# Autodesk Inventor assembly: BaffleAssembly2
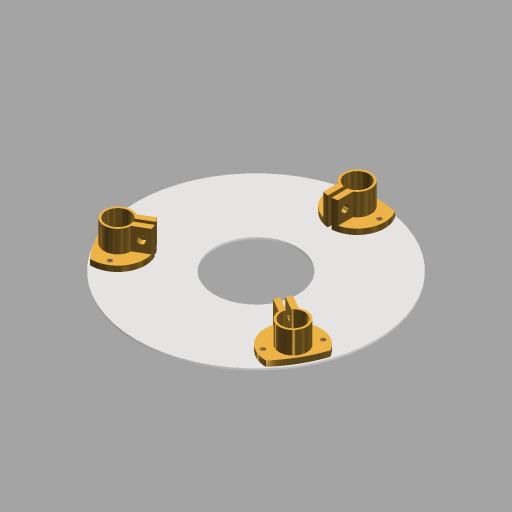
[picture p0: Inventor's stored thumbnail of the model, 512x512]
Saved by Autodesk Inventor 2024 (Build 280153020, 153B)
## iProperties
Created: 2023-10-26
Part Number: BaffleAssembly2
Document SubType Name: Assembly
Designer: schanen
Mass: 44.3536 g
Surface Area: 289.72 cm^2
Volume: 15.1113 cm^3
Density: 2.93513 g/cm^3
Author: schanen
## Documents named in this file (3)
- C:\Users\schanen\Documents\Inventor\LargeTransportDewarInsert2023\BaffleAssembly2.iam
- C:\Users\schanen\Documents\Inventor\LargeTransportDewarInsert2023\Baffle.ipt
- C:\Users\schanen\Documents\Inventor\LargeTransportDewarInsert2023\BaffleClampWithScrew.ipt
## Components (4 placed, 2 different names)
1. Baffle:1 — Mate:1, Mate:2, Mate:3
2. BaffleClampWithScrew:1 [sub-assembly] — Mate:1, Mate:2, Mate:3
3. BaffleClampWithScrew:2 [sub-assembly]
4. BaffleClampWithScrew:3 [sub-assembly]
## Component patterns: (3 elements, first: BaffleClampWithScrew:1)
## Relationships (3: Mate 3)
- Mate:1: Baffle:1 ↔ BaffleClampWithScrew:1
- Mate:2: Baffle:1 ↔ BaffleClampWithScrew:1
- Mate:3: Baffle:1 ↔ BaffleClampWithScrew:1
